# Autodesk Inventor assembly: tension
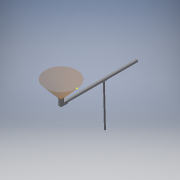
[picture p0: Inventor's stored thumbnail of the model, 180x180]
Saved by Autodesk Inventor 2018 (Build 220112000, 112)
## iProperties
Created: 2020-04-19
Part Number: tension
Document SubType Name: Assembly
Designer: Darshan
Author: Darshan
## Documents named in this file (5)
- E:\tension.iam
- C:\Users\Darshan\Pictures\expofunl2.ipt
- C:\Users\Darshan\Pictures\elbow3_CPY.ipt
- C:\Users\Darshan\Pictures\expopipe.ipt
- C:\Users\Darshan\Pictures\Assembly5.iam
## Components (4 placed, 4 different names)
1. expofunl2:1 — Rigid:1
2. elbow3_CPY:1 — Rigid:1, Rigid:2
3. expopipe:1 — Rigid:2, Rigid:3
4. Assembly5:1 [sub-assembly] — Rigid:3
## Relationships (3: WeldJoint 3)
- Rigid:1 [WeldJoint]: expofunl2:1 ↔ elbow3_CPY:1
- Rigid:2 [WeldJoint]: elbow3_CPY:1 ↔ expopipe:1
- Rigid:3 [WeldJoint]: expopipe:1 ↔ Assembly5:1
